# Autodesk Inventor assembly: lw_6_сборка_2
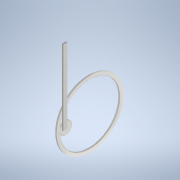
[picture p0: Inventor's stored thumbnail of the model, 180x180]
Saved by Autodesk Inventor 2021 (Build 250183000, 183)
## iProperties
Created: 2021-05-17
Part Number: lw_6_сборка_2
Document SubType Name: Assembly
Designer: davam
Author: davam
## Documents named in this file (3)
- C:\Users\davam\Desktop\лаб_6\lw_6_сборка_2.iam
- C:\Users\davam\Desktop\лаб_6\lw_6_сборка_2\Мастер проектирования\Цилиндрическое зубчатое зацепление1.iam
- C:\Users\davam\Desktop\лаб_6\lw_6_part3.ipt
## Components (2 placed, 2 different names)
1. Цилиндрическое зубчатое зацепление:1 [sub-assembly] — Совмещение:1, Совмещение:2, Угол:1
2. lw_6_part3:1 — Совмещение:1, Совмещение:2, Угол:1
## Relationships (3: Mate 2, Angle 1)
- Совмещение:1 [Mate]: Цилиндрическое зубчатое зацепление:1 ↔ lw_6_part3:1
- Совмещение:2 [Mate]: Цилиндрическое зубчатое зацепление:1 ↔ lw_6_part3:1
- Угол:1 [Angle] (90 deg): Цилиндрическое зубчатое зацепление:1 ↔ lw_6_part3:1
